# Autodesk Inventor assembly: innerHorn slider
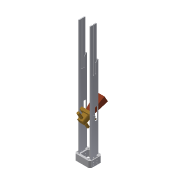
[picture p0: Inventor's stored thumbnail of the model, 180x180]
Saved by Autodesk Inventor 2015 SP1 (Build 190203100, 203)
## iProperties
Created: 2016-04-08
Part Number: innerHorn slider
Document SubType Name: Assembly
Designer: jad211
Author: jad211
## Documents named in this file (7)
- C:\ColdMatter\CADFiles\EDM Machine\Detection Region\Microwave Horn Assembly\innerHorn slider.iam
- C:\ColdMatter\CADFiles\EDM Machine\Detection Region\Microwave Horn Assembly\Horn with Flange.iam
- C:\ColdMatter\CADFiles\EDM Machine\Detection Region\Microwave Horn Assembly\Horn support.ipt
- C:\ColdMatter\CADFiles\EDM Machine\Pumping Region\coaxToWaveguidWG18.ipt
- C:\ColdMatter\CADFiles\EDM Machine\Detection Region\Microwave Horn Assembly\rod.ipt
- C:\ColdMatter\CADFiles\EDM Machine\Detection Region\Microwave Horn Assembly\DN63CF blank With Holes.ipt
- C:\ColdMatter\CADFiles\EDM Machine\Detection Region\Microwave Horn Assembly\supportHolder.ipt
## Components (10 placed, 6 different names)
1. Horn with Flange:1 [sub-assembly] — Mate:35, Angle:1, Mate:36, Mate:37, Mate:38, Mate:39, Mate:40, Mate:41, Mate:42, Mate:43, Mate:44, Mate:45, Mate:46
2. Horn support:1 — Mate:50, Mate:51
3. Horn support:2 — Mate:47, Mate:48, Mate:53, Mate:54
4. coaxToWaveguidWG18:1 — Mate:34, Mate:36, Mate:37, Mate:38
5. rod:1 — Mate:45, Mate:46
6. rod:2 — Mate:43, Mate:44, Mate:51
7. rod:4 — Mate:39, Mate:40, Mate:48
8. DN63CF blank With Holes:1 — Flush:5
9. rod:5 — Tangent:1, Mate:41, Mate:42
10. supportHolder:1 — Mate:52, Mate:53, Mate:54
## Relationships (23: Mate 20, Flush 1, Tangent 1, Angle 1)
- Flush:5: DN63CF blank With Holes:1
- Tangent:1: rod:5
- Mate:34: coaxToWaveguidWG18:1
- Mate:35: Horn with Flange:1
- Angle:1 (120 deg): Horn with Flange:1
- Mate:36: Horn with Flange:1 ↔ coaxToWaveguidWG18:1
- Mate:37: Horn with Flange:1 ↔ coaxToWaveguidWG18:1
- Mate:38: Horn with Flange:1 ↔ coaxToWaveguidWG18:1
- Mate:39: Horn with Flange:1 ↔ rod:4
- Mate:40: Horn with Flange:1 ↔ rod:4
- Mate:41: Horn with Flange:1 ↔ rod:5
- Mate:42: Horn with Flange:1 ↔ rod:5
- Mate:43: Horn with Flange:1 ↔ rod:2
- Mate:44: Horn with Flange:1 ↔ rod:2
- Mate:45: Horn with Flange:1 ↔ rod:1
- Mate:46: Horn with Flange:1 ↔ rod:1
- Mate:47: Horn support:2
- Mate:48: Horn support:2 ↔ rod:4
- Mate:50: Horn support:1
- Mate:51: Horn support:1 ↔ rod:2
- Mate:52: supportHolder:1
- Mate:53: Horn support:2 ↔ supportHolder:1
- Mate:54: Horn support:2 ↔ supportHolder:1
